# Autodesk Inventor assembly: tendon_wh_2_ass
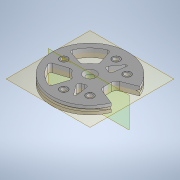
[picture p0: Inventor's stored thumbnail of the model, 180x180]
Saved by Autodesk Inventor 2020 (Build 240168000, 168)
## iProperties
Created: 2020-12-12
Part Number: tendon_wh_2_ass
Document SubType Name: Assembly
Designer: Shuang Peng
Author: Shuang Peng
## Documents named in this file (3)
- D:\projects-3\biped_tiny\hardware\tendon_wh_2_ass.iam
- D:\projects-3\biped_tiny\hardware\tendon_wh_2.ipt
- D:\projects-3\biped_tiny\hardware\screw_holder_2_3.ipt
## Components (6 placed, 2 different names)
1. tendon_wh_2:1 — Insert:1, Insert:2, Insert:3, Insert:4, Insert:5
2. screw_holder_2_3:1 — Insert:1
3. screw_holder_2_3:2 — Insert:2
4. screw_holder_2_3:3 — Insert:3
5. screw_holder_2_3:4 — Insert:4
6. screw_holder_2_3:5 — Insert:5
## Relationships (5: Insert 5)
- Insert:1: tendon_wh_2:1 ↔ screw_holder_2_3:1
- Insert:2: tendon_wh_2:1 ↔ screw_holder_2_3:2
- Insert:3: tendon_wh_2:1 ↔ screw_holder_2_3:3
- Insert:4: tendon_wh_2:1 ↔ screw_holder_2_3:4
- Insert:5: tendon_wh_2:1 ↔ screw_holder_2_3:5
